# Autodesk Inventor assembly: 2421-c2421-20
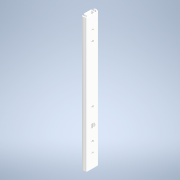
[picture p0: Inventor's stored thumbnail of the model, 180x180]
Saved by Autodesk Inventor 2021 (Build 250183000, 183)
## iProperties
Created: 2017-06-19
Part Number: 2421-c2421-20
Document SubType Name: Assembly
Designer: Hagihara Yuya
Sending System: spGate
Preprocessor: spGate 11.3.14
Title: C2421_20_3D.stp
## Documents named in this file (3)
- C:\Users\Hagihara Yuya\Documents\GrabCAD\NHK2021\BasicParts\よく使う部品（萩原）\SlideRail\2421-c2421-20\2421-c2421-20.iam
- C:\Users\Hagihara Yuya\Documents\GrabCAD\NHK2021\BasicParts\よく使う部品（萩原）\SlideRail\2421-c2421-20\C2421_20_3D-prt0.ipt
- C:\Users\Hagihara Yuya\Documents\GrabCAD\NHK2021\BasicParts\よく使う部品（萩原）\SlideRail\2421-c2421-20\C2421_20_3D-prt1.ipt
## Components (2 placed, 2 different names)
1. C2421_20_3D-prt0 — スライダ:1
2. C2421_20_3D-prt1 — スライダ:1
## Relationships (1: TranslationJoint 1)
- スライダ:1 [TranslationJoint] (6.48 mm): C2421_20_3D-prt0 ↔ C2421_20_3D-prt1
